# Autodesk Inventor assembly: Лестница СБ
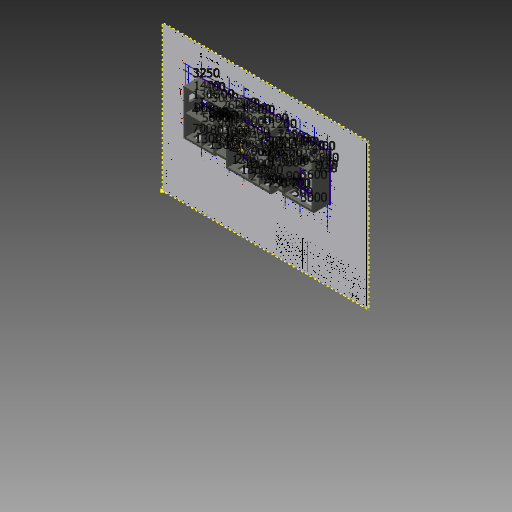
[picture p0: Inventor's stored thumbnail of the model, 512x512]
Saved by Autodesk Inventor 2019 (Build 230136000, 136)
## iProperties
Created: 2018-10-10
Part Number: Лестница СБ
Material: Типовые
Document SubType Name: Assembly
Designer: Андреев Н.Л.
Mass: 2.69693e+08 g
Surface Area: 1.09391e+07 cm^2
Volume: 1.54669e+08 cm^3
Density: 1.74367 g/cm^3
пПодъемов: 20,0 бр
пПодъем: 163
пХод: 296,8 мм
пЭффШаг: 621,8 мм
пСвес: 30,2 мм
пТолПроступи: 40,0 мм
пТолКосоура: 40,0 мм
пТолСтолба: 90,0 мм
пТолБалясины: 40,0 мм
пШирКосоура: 300,0 мм
зУр2Эт: 3250,0 мм
зДл: 3000,0 мм
зШир: 2000,0 мм
пДлПроступи: 900,0 мм
пШирПроступи: 327,0 мм
Author: Андреев Н.Л.
## Documents named in this file (5)
- C:\Users\andrnl\Documents\Inventor\Мурзин\Лестница СБ.iam
- C:\Users\andrnl\Documents\Inventor\Мурзин\Этаж 1.ipt
- C:\Users\andrnl\Documents\Inventor\Мурзин\Лестница.iam
- C:\Users\andrnl\Documents\Inventor\Мурзин\Перекрытие коридора.ipt
- C:\Users\andrnl\Documents\Inventor\Мурзин\Лестница Мурзин.xlsx
## Components (3 placed, 3 different names)
1. Этаж 1:1 — Совмещение:1, Совмещение:2, Заподлицо:2
2. Лестница:1 [sub-assembly] — Совмещение:1, Совмещение:2, Заподлицо:1
3. Перекрытие коридора:1 — Заподлицо:2
## Relationships (4: Mate 2, Flush 2)
- Совмещение:1 [Mate]: Этаж 1:1 ↔ Лестница:1
- Совмещение:2 [Mate]: Этаж 1:1 ↔ Лестница:1
- Заподлицо:1 [Flush]: Лестница:1
- Заподлицо:2 [Flush]: Этаж 1:1 ↔ Перекрытие коридора:1
## Named parameters: зУр2Эт = 3250 mm, зДл = 3000 mm, зШир = 2000 mm, пДлПроступи = 900 mm, пПодъемов = 20, пПодъем = 162.5 mm, пХод = 296.8 mm, пЭффШаг = 621.8 mm, пСвес = 30.2 mm, пТолПроступи = 40 mm, пТолКосоура = 40 mm, пТолСтолба = 90 mm, пТолБалясины = 40 mm, пШирКосоура = 300 mm, пОтступСтен = 5 mm, пДиаг = 338.3733 mm, пПлощадка = 1, пПодъемов2 = 7, пВыход2Ур = 1, пПодъемов1 = 11, пШирПроступи = 327 mm, пТолПодступенка = 17.4 mm, пШипПодступ = 10 mm, пОтступШипа = 50 mm, пГлубПаза = 12 mm, пОтступПодступ = 10 mm, пОтступОтСтен = 5 mm, пДлПлощадки = 1990 mm, пТолПричала = 17.4 mm, зТолПерекрытия = 300 mm, пСвесВбок = 30 mm
